# Autodesk Inventor assembly: 446 FIRST HiGrip Wheel Shaft
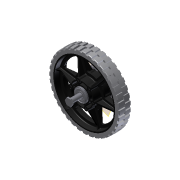
[picture p0: Inventor's stored thumbnail of the model, 180x180]
Saved by Autodesk Inventor 2013 (Build 170138000, 138)
## iProperties
Created: 2012-10-14
Part Number: 446 FIRST HiGrip Wheel Shaft
Document SubType Name: Assembly
Designer: Nemo
Mass: 338.876 g
Surface Area: 1139.75 cm^2
Volume: 205.855 cm^3
Density: 1.64619 g/cm^3
Author: Nemo
## Documents named in this file (7)
- H:\Nemo\Documents\Robotics\COTS Parts\Gearboxes\Shafts\446 FIRST HiGrip Wheel Shaft.iam
- H:\Nemo\Documents\Robotics\COTS Parts\Wheels\6in FIRST Wheel 2012 HiGrip.iam
- H:\Nemo\Documents\Robotics\COTS Parts\Gearboxes\Bearings\Bearing 1614zz.ipt
- H:\Nemo\Documents\Robotics\COTS Parts\Fasteners\38-16 hexbolt x3500.ipt
- H:\Nemo\Documents\Robotics\COTS Parts\Fasteners\38-16 locknut.ipt
- H:\Nemo\Documents\Robotics\COTS Parts\Gearboxes\Spacers\446 wheel sprocket spacer.ipt
- H:\Nemo\Documents\Robotics\COTS Parts\Sprockets\25 sprocket 32T.ipt
## Components (7 placed, 6 different names)
1. 6in FIRST Wheel 2012 HiGrip:1 [sub-assembly] — Insert:1, Insert:2, Mate:5, Mate:6, Mate:7
2. Bearing 1614zz:1 — Insert:1, Mate:1
3. Bearing 1614zz:2 — Insert:2, Mate:8
4. 38-16 hexbolt x3500:1 — Mate:1, Mate:2, Mate:3, Mate:4
5. 38-16 locknut:1 — Mate:2, Mate:3
6. 446 wheel sprocket spacer:1 — Mate:4, Mate:8
7. 25 Sprocket 32T:1 — Mate:5, Mate:6, Mate:7
## Relationships (10: Mate 8, Insert 2)
- Insert:1: 6in FIRST Wheel 2012 HiGrip:1 ↔ Bearing 1614zz:1
- Insert:2: 6in FIRST Wheel 2012 HiGrip:1 ↔ Bearing 1614zz:2
- Mate:1: Bearing 1614zz:1 ↔ 38-16 hexbolt x3500:1
- Mate:2: 38-16 hexbolt x3500:1 ↔ 38-16 locknut:1
- Mate:3 (72.39 mm): 38-16 hexbolt x3500:1 ↔ 38-16 locknut:1
- Mate:4: 38-16 hexbolt x3500:1 ↔ 446 wheel sprocket spacer:1
- Mate:5: 6in FIRST Wheel 2012 HiGrip:1 ↔ 25 Sprocket 32T:1
- Mate:6: 6in FIRST Wheel 2012 HiGrip:1 ↔ 25 Sprocket 32T:1
- Mate:7: 6in FIRST Wheel 2012 HiGrip:1 ↔ 25 Sprocket 32T:1
- Mate:8: Bearing 1614zz:2 ↔ 446 wheel sprocket spacer:1
